# Autodesk Inventor assembly: CMV12000 Extraction Tool V02
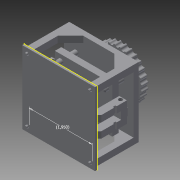
[picture p0: Inventor's stored thumbnail of the model, 180x180]
Saved by Autodesk Inventor 2015 (Build 190159000, 159)
## iProperties
Created: 2016-09-16
Part Number: CMV12000 Extraction Tool V02
Document SubType Name: Assembly
Designer: spichelh
Author: spichelh
## Documents named in this file (7)
- C:\Users\spichelh\Documents\GitHub\beta-hardware\Manufacturing Tools\CMV12000 Extraction Tool V01\CMV12000 Extraction Tool V02.iam
- C:\Users\spichelh\Documents\GitHub\beta-hardware\Manufacturing Tools\CMV12000 Extraction Tool V01\CMV12000v1.ipt
- C:\Users\spichelh\Documents\GitHub\beta-hardware\Manufacturing Tools\CMV12000 Extraction Tool V01\base.ipt
- C:\Users\spichelh\Documents\GitHub\beta-hardware\Manufacturing Tools\CMV12000 Extraction Tool V01\SFE PCB.ipt
- C:\Users\spichelh\Documents\GitHub\beta-hardware\Manufacturing Tools\CMV12000 Extraction Tool V01\mover02.ipt
- C:\Users\spichelh\Documents\GitHub\beta-hardware\Manufacturing Tools\CMV12000 Extraction Tool V01\arms02.ipt
- C:\Users\spichelh\Documents\GitHub\beta-hardware\Manufacturing Tools\CMV12000 Extraction Tool V01\Knob02.ipt
## Components (9 placed, 6 different names)
1. CMV12000v1:1 — Flush:8, Flush:9, Mate:7, Mate:15
2. arms02:2 — Rotational:1
3. arms02:3 — Rotational:4
4. base:1 — Flush:8, Flush:9, Mate:7, Mate:8, Mate:9, Mate:10, Mate:12, Mate:20, Mate:21, Mate:22
5. arms02:1 — Rotational:2
6. arms02:4 — Rotational:3
7. mover02:1 — Mate:8, Mate:9, Mate:10, Rotational:1, Rotational:2, Rotational:3, Rotational:4
8. Knob02:1 — Mate:12
9. SFE PCB:1 — Mate:15, Mate:18, Mate:19, Flush:10, Mate:20, Mate:21, Mate:22
## Relationships (18: Mate 11, RevoluteJoint 4, Flush 3)
- Flush:8 (-3 mm): CMV12000v1:1 ↔ base:1
- Flush:9 (-1 mm): CMV12000v1:1 ↔ base:1
- Mate:7 (5.365 mm): CMV12000v1:1 ↔ base:1
- Mate:8: base:1 ↔ mover02:1
- Mate:9: base:1 ↔ mover02:1
- Mate:10 (7 mm): base:1 ↔ mover02:1
- Mate:12: base:1 ↔ Knob02:1
- Mate:15 (4 mm): CMV12000v1:1 ↔ SFE PCB:1
- Mate:18: SFE PCB:1
- Mate:19: SFE PCB:1
- Flush:10: SFE PCB:1
- Mate:20: base:1 ↔ SFE PCB:1
- Mate:21: base:1 ↔ SFE PCB:1
- Rotational:1 [RevoluteJoint]: arms02:2 ↔ mover02:1
- Rotational:2 [RevoluteJoint]: arms02:1 ↔ mover02:1
- Rotational:3 [RevoluteJoint]: arms02:4 ↔ mover02:1
- Rotational:4 [RevoluteJoint]: arms02:3 ↔ mover02:1
- Mate:22: base:1 ↔ SFE PCB:1
